# Autodesk Inventor assembly: CE-9.1.3
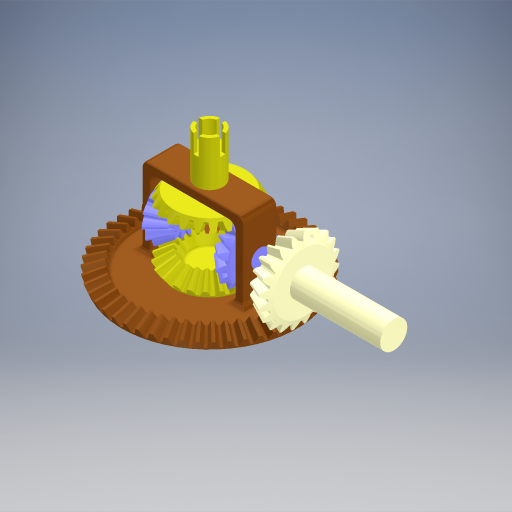
[picture p0: Inventor's stored thumbnail of the model, 512x512]
Saved by Autodesk Inventor 2024 (Build 280153000, 153)
## iProperties
Created: 2024-03-14
Part Number: CE-9.1.3
Document SubType Name: Assembly
Designer: Alex
Author: Alex
## Documents named in this file (5)
- C:\Shared\alex-bartella-schoolwork\4z03\Week 9\CE-9.1.3.iam
- C:\Shared\alex-bartella-schoolwork\4z03\Week 9\STEP\CE-9.1.3 STEP Files\Cage\Cage.ipt
- C:\Shared\alex-bartella-schoolwork\4z03\Week 9\STEP\CE-9.1.3 STEP Files\Driver\Driver.ipt
- C:\Shared\alex-bartella-schoolwork\4z03\Week 9\STEP\CE-9.1.3 STEP Files\Ring\Ring.ipt
- C:\Shared\alex-bartella-schoolwork\4z03\Week 9\STEP\CE-9.1.3 STEP Files\Sun\Sun.ipt
## Components (6 placed, 4 different names)
1. Cage:1 — Mate:9, Mate:10, Rotation:2, Rotation:3, Rotation:4
2. Cage:2 — Mate:8, Mate:11, Rotation:4
3. Driver:1 — Mate:6, Flush:2, Driver, Rotation:1
4. Ring:1 — Flush:1, Mate:2, Mate:3, Mate:5, Mate:7, Rotation:1, Mate:8, Mate:9, Mate:10, Mate:11
5. Sun:1 — Mate:2, Mate:5, Mate:4, Rotation:2, Driver_top
6. Sun:2 — Mate:3, Mate:4, Rotation:3
## Relationships (18: Mate 10, RelateRotation 4, Flush 2, Angle 2)
- Flush:1: Ring:1
- Mate:2: Ring:1 ↔ Sun:1
- Mate:3: Ring:1 ↔ Sun:2
- Mate:4 (-38 mm): Sun:1 ↔ Sun:2
- Mate:5: Ring:1 ↔ Sun:1
- Mate:6: Driver:1
- Mate:7: Ring:1
- Flush:2 (52 mm): Driver:1
- Driver [Angle] (0 deg): Driver:1
- Rotation:1 [RelateRotation] (0.4 ul): Driver:1 ↔ Ring:1
- Mate:8: Cage:2 ↔ Ring:1
- Mate:9: Cage:1 ↔ Ring:1
- Mate:10: Cage:1 ↔ Ring:1
- Mate:11: Cage:2 ↔ Ring:1
- Rotation:2 [RelateRotation] (0.6818 ul): Cage:1 ↔ Sun:1
- Rotation:3 [RelateRotation] (0.6818 ul): Cage:1 ↔ Sun:2
- Rotation:4 [RelateRotation] (1 ul): Cage:1 ↔ Cage:2
- Driver_top [Angle] (0 deg): Sun:1
